# Autodesk Inventor assembly: L3 Gearbox Assembly
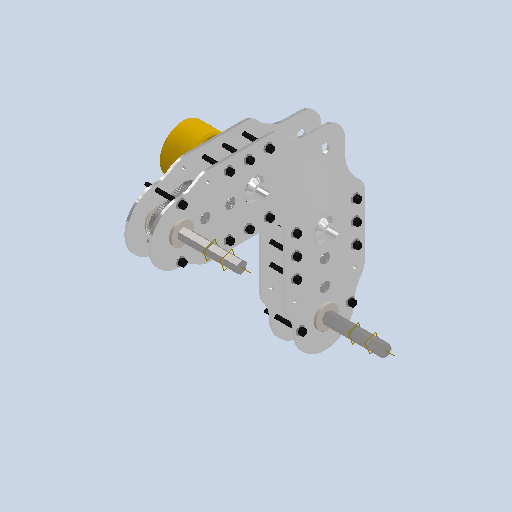
[picture p0: Inventor's stored thumbnail of the model, 512x512]
Saved by Autodesk Inventor 2025.1 (Build 291241020, 241B)
## iProperties
Created: 2023-02-14
Part Number: L3 Gearbox Assembly
Document SubType Name: Assembly
Designer: Dave
Mass: 1965.41 g
Surface Area: 3646.76 cm^2
Volume: 537.619 cm^3
Density: 3.65577 g/cm^3
Author: Dave
## Documents named in this file (15)
- C:\Users\t205b\OneDrive\Documents\Github\BehrendURCMechanical\CAD\Chassis V3\L3 Gearbox Assembly.iam
- C:\Users\t205b\OneDrive\Documents\Github\BehrendURCMechanical\CAD\Chassis\GearBox\Final Gears and Assemblies\CH-1-01-20T_Drive Gear.ipt
- C:\Users\t205b\OneDrive\Documents\Github\BehrendURCMechanical\CAD\Chassis\GearBox\Final Gears and Assemblies\CH-1-01-60T_Output.ipt
- C:\Users\t205b\OneDrive\Documents\Github\BehrendURCMechanical\CAD\Chassis\GearBox\Final Gears and Assemblies\CH-1-01-20T_Idler.ipt
- C:\Users\t205b\OneDrive\Documents\Github\BehrendURCMechanical\CAD\Chassis\GearBox\Final Gears and Assemblies\CH-1-01-60T_Idler.ipt
- C:\Users\t205b\OneDrive\Documents\Github\BehrendURCMechanical\CAD\Chassis\GearBox\Drive Motor Shaft Coupler.ipt
- C:\Users\t205b\OneDrive\Documents\Github\BehrendURCMechanical\CAD\Chassis\GearBox\Ch-1-01-0.5x4.5HexShaft.ipt
- C:\Users\t205b\OneDrive\Documents\Github\BehrendURCMechanical\CAD\Chassis\GearBox\CH-1-01-0.25x1.875SmoothShaft.ipt
- C:\Users\t205b\OneDrive\Documents\Github\BehrendURCMechanical\CAD\Chassis\GearBox\CH-1-01-0.5HexBearing.ipt
- C:\Users\t205b\OneDrive\Documents\Github\BehrendURCMechanical\CAD\Chassis\GearBox\CH-1-01-0.25IDSmoothBoreBearing.ipt
- C:\Users\t205b\OneDrive\Documents\Github\BehrendURCMechanical\CAD\Chassis V3\DriveMotorAssem\DriveMotorAssem.iam
- C:\Users\t205b\OneDrive\Documents\Github\BehrendURCMechanical\CAD\Chassis V3\91251A252_Black-Oxide Alloy Steel Socket Head Screw.ipt
- C:\Users\Dave\Downloads\91831A011_18-8 Stainless Steel Nylon-Insert Locknut (1).ipt
- C:\Users\t205b\OneDrive\Documents\Github\BehrendURCMechanical\CAD\Chassis V3\90107A011_316 Stainless Steel Washer.ipt
- C:\Users\t205b\OneDrive\Documents\Github\BehrendURCMechanical\CAD\Chassis V3\L3Plate.ipt
## Components (99 placed, 14 different names)
1. L3Plate:1 — Insert:13, Insert:14, Insert:15, Insert:16, Insert:17, Insert:18, Insert:19, Insert:20
2. L3Plate:2 — Mate:29, Insert:39, Insert:41
3. CH-1-01-0.25IDSmoothBoreBearing:4 — Mate:10, Mate:21
4. DriveMotorAssem:1 [sub-assembly] — Mate:27, Insert:21, Insert:22, Insert:23, Insert:24, Insert:25, Insert:26, Mate:29, Mate:30, Mate:31
5. 91831A011_18-8 Stainless Steel Nylon-Insert Locknut (1):4 — Insert:36
6. 91251A252_Black-Oxide Alloy Steel Socket Head Screw:1 — Insert:27, Mate:31
7. 90107A011_316 Stainless Steel Washer:1 — Insert:23, Insert:36
8. 91831A011_18-8 Stainless Steel Nylon-Insert Locknut (1):3 — Insert:37
9. 90107A011_316 Stainless Steel Washer:4 — Insert:22, Insert:37
10. 91251A252_Black-Oxide Alloy Steel Socket Head Screw:2 — Insert:28
11. 90107A011_316 Stainless Steel Washer:6 — Insert:21, Insert:38
12. 91251A252_Black-Oxide Alloy Steel Socket Head Screw:5 — Insert:30
13. 91831A011_18-8 Stainless Steel Nylon-Insert Locknut (1):2 — Insert:38
14. 91251A252_Black-Oxide Alloy Steel Socket Head Screw:6 — Insert:33
15. 91831A011_18-8 Stainless Steel Nylon-Insert Locknut (1):5 — Insert:42
16. 90107A011_316 Stainless Steel Washer:12 — Insert:24, Insert:42
17. 91251A252_Black-Oxide Alloy Steel Socket Head Screw:7 — Insert:34
18. 91831A011_18-8 Stainless Steel Nylon-Insert Locknut (1):6 — Insert:43
19. 90107A011_316 Stainless Steel Washer:14 — Insert:25, Insert:43
20. 91251A252_Black-Oxide Alloy Steel Socket Head Screw:8 — Insert:35
21. 91831A011_18-8 Stainless Steel Nylon-Insert Locknut (1):8 — Insert:44
22. 90107A011_316 Stainless Steel Washer:16 — Insert:26, Insert:44
23. 91251A252_Black-Oxide Alloy Steel Socket Head Screw:4 — Insert:32
24. 91831A011_18-8 Stainless Steel Nylon-Insert Locknut (1):7 — Insert:40
25. 90107A011_316 Stainless Steel Washer:10 — Insert:40, Insert:41
26. 91251A252_Black-Oxide Alloy Steel Socket Head Screw:3 — Insert:31
27. 91831A011_18-8 Stainless Steel Nylon-Insert Locknut (1):1 — Insert:45
28. 90107A011_316 Stainless Steel Washer:8 — Insert:39, Insert:45
29. CH-1-01-0.5HexBearing:1 — Mate:17, Flush:8
30. Ch-1-01-0.5x4.5HexShaft:1 — Mate:8, Mate:9, Flush:8
31. CH-1-01-0.25IDSmoothBoreBearing:3 — Flush:4, Mate:18, Mate:20, Mate:22, Mate:28
32. CH-1-01-0.25x1.875SmoothShaft:2 — Insert:12, Flush:4, Mate:28
33. Drive Motor Shaft Coupler:1 — Mate:27, Mate:30, Insert:29
34. CH-1-01-0.25IDSmoothBoreBearing:2 — Mate:11
35. CH-1-01-0.25x1.875SmoothShaft:1
36. CH-1-01-0.25IDSmoothBoreBearing:1 — Insert:12
37. CH-1-01-0.5HexBearing:2 — Mate:8, Mate:9
38. CH-1-01-20T_Drive Gear:1 — Insert:29
39. CH-1-01-60T_Idler:2 — Mate:10, Mate:11
40. CH-1-01-20T_Idler:1 — Mate:21, Flush:5
41. CH-1-01-60T_Idler:1 — Mate:18, Mate:19, Mate:20, Flush:5
42. CH-1-01-20T_Idler:2 — Mate:19, Mate:22, Flush:6
43. CH-1-01-60T_Output:1 — Mate:17, Flush:6
44. 90107A011_316 Stainless Steel Washer:11 — Insert:18, Insert:33
45. 90107A011_316 Stainless Steel Washer:13 — Insert:19, Insert:34
46. 90107A011_316 Stainless Steel Washer:15 — Insert:20, Insert:35
47. 90107A011_316 Stainless Steel Washer:9 — Insert:17, Insert:32
48. 90107A011_316 Stainless Steel Washer:7 — Insert:16, Insert:31
49. 90107A011_316 Stainless Steel Washer:5 — Insert:15, Insert:30
50. 90107A011_316 Stainless Steel Washer:3 — Insert:14, Insert:28
51. 90107A011_316 Stainless Steel Washer:2 — Insert:13, Insert:27
52. DriveMotorAssem:2 [sub-assembly]
53. 91831A011_18-8 Stainless Steel Nylon-Insert Locknut (1):9
54. 91251A252_Black-Oxide Alloy Steel Socket Head Screw:9
55. 90107A011_316 Stainless Steel Washer:17
56. 91831A011_18-8 Stainless Steel Nylon-Insert Locknut (1):10
57. 90107A011_316 Stainless Steel Washer:18
58. 91251A252_Black-Oxide Alloy Steel Socket Head Screw:10
59. 90107A011_316 Stainless Steel Washer:19
60. 91251A252_Black-Oxide Alloy Steel Socket Head Screw:11
61. 91831A011_18-8 Stainless Steel Nylon-Insert Locknut (1):11
62. 91251A252_Black-Oxide Alloy Steel Socket Head Screw:12
63. 91831A011_18-8 Stainless Steel Nylon-Insert Locknut (1):12
64. 90107A011_316 Stainless Steel Washer:20
65. 91251A252_Black-Oxide Alloy Steel Socket Head Screw:13
66. 91831A011_18-8 Stainless Steel Nylon-Insert Locknut (1):13
67. 90107A011_316 Stainless Steel Washer:21
68. 91251A252_Black-Oxide Alloy Steel Socket Head Screw:14
69. 91831A011_18-8 Stainless Steel Nylon-Insert Locknut (1):14
70. 90107A011_316 Stainless Steel Washer:22
71. 91251A252_Black-Oxide Alloy Steel Socket Head Screw:15
72. 91831A011_18-8 Stainless Steel Nylon-Insert Locknut (1):15
73. 90107A011_316 Stainless Steel Washer:23
74. 91251A252_Black-Oxide Alloy Steel Socket Head Screw:16
75. 91831A011_18-8 Stainless Steel Nylon-Insert Locknut (1):16
76. 90107A011_316 Stainless Steel Washer:24
77. CH-1-01-0.5HexBearing:3
78. Ch-1-01-0.5x4.5HexShaft:2
79. CH-1-01-0.25IDSmoothBoreBearing:5
80. CH-1-01-0.25x1.875SmoothShaft:3
81. Drive Motor Shaft Coupler:2
82. CH-1-01-0.25IDSmoothBoreBearing:6
83. CH-1-01-0.25x1.875SmoothShaft:4
84. CH-1-01-0.25IDSmoothBoreBearing:7
85. CH-1-01-0.5HexBearing:4
86. CH-1-01-20T_Drive Gear:2
87. CH-1-01-60T_Idler:3
88. CH-1-01-20T_Idler:3
89. CH-1-01-60T_Idler:4
90. CH-1-01-20T_Idler:4
91. CH-1-01-60T_Output:2
92. 90107A011_316 Stainless Steel Washer:25
93. 90107A011_316 Stainless Steel Washer:26
94. 90107A011_316 Stainless Steel Washer:27
95. 90107A011_316 Stainless Steel Washer:28
96. 90107A011_316 Stainless Steel Washer:29
97. 90107A011_316 Stainless Steel Washer:30
98. 90107A011_316 Stainless Steel Washer:31
99. 90107A011_316 Stainless Steel Washer:32
## Component patterns: (2 elements, first: DriveMotorAssem:1 + 91831A011_18-8 Stainless Steel Nylon-Insert Locknut (1):4 + 91251A252_Black-Oxide Alloy Steel Socket Head Screw:1 + 90107A011_316 Stainless Steel Washer:1 + 91831A011_18-8 Stainless Steel Nylon-Insert Locknut (1):3 + 90107A011_316 Stainless Steel Washer:4 + 91251A252_Black-Oxide Alloy Steel Socket Head Screw:2 + 90107A011_316 Stainless Steel Washer:6 + 91251A252_Black-Oxide Alloy Steel Socket Head Screw:5 + 91831A011_18-8 Stainless Steel Nylon-Insert Locknut (1):2 + 91251A252_Black-Oxide Alloy Steel Socket Head Screw:6 + 91831A011_18-8 Stainless Steel Nylon-Insert Locknut (1):5 + 90107A011_316 Stainless Steel Washer:12 + 91251A252_Black-Oxide Alloy Steel Socket Head Screw:7 + 91831A011_18-8 Stainless Steel Nylon-Insert Locknut (1):6 + 90107A011_316 Stainless Steel Washer:14 + 91251A252_Black-Oxide Alloy Steel Socket Head Screw:8 + 91831A011_18-8 Stainless Steel Nylon-Insert Locknut (1):8 + 90107A011_316 Stainless Steel Washer:16 + 91251A252_Black-Oxide Alloy Steel Socket Head Screw:4 + 91831A011_18-8 Stainless Steel Nylon-Insert Locknut (1):7 + 90107A011_316 Stainless Steel Washer:10 + 91251A252_Black-Oxide Alloy Steel Socket Head Screw:3 + 91831A011_18-8 Stainless Steel Nylon-Insert Locknut (1):1 + 90107A011_316 Stainless Steel Washer:8 + CH-1-01-0.5HexBearing:1 + Ch-1-01-0.5x4.5HexShaft:1 + CH-1-01-0.25IDSmoothBoreBearing:3 + CH-1-01-0.25x1.875SmoothShaft:2 + Drive Motor Shaft Coupler:1 + CH-1-01-0.25IDSmoothBoreBearing:2 + CH-1-01-0.25x1.875SmoothShaft:1 + CH-1-01-0.25IDSmoothBoreBearing:1 + CH-1-01-0.5HexBearing:2 + CH-1-01-20T_Drive Gear:1 + CH-1-01-60T_Idler:2 + CH-1-01-20T_Idler:1 + CH-1-01-60T_Idler:1 + CH-1-01-20T_Idler:2 + CH-1-01-60T_Output:1 + 90107A011_316 Stainless Steel Washer:11 + 90107A011_316 Stainless Steel Washer:13 + 90107A011_316 Stainless Steel Washer:15 + 90107A011_316 Stainless Steel Washer:9 + 90107A011_316 Stainless Steel Washer:7 + 90107A011_316 Stainless Steel Washer:5 + 90107A011_316 Stainless Steel Washer:3 + 90107A011_316 Stainless Steel Washer:2)
## Relationships (62: Insert 40, Mate 16, Flush 5, Angle 1)
- [Angle] (0 deg): L3Plate:1
- [Flush]: L3Plate:1 ↔ L3Plate:2
- [Insert]: L3Plate:1 ↔ CH-1-01-0.25IDSmoothBoreBearing:1
- [Insert]: L3Plate:1 ↔ CH-1-01-0.25IDSmoothBoreBearing:2
- [Insert]: L3Plate:2 ↔ CH-1-01-0.25IDSmoothBoreBearing:3
- [Insert]: L3Plate:2 ↔ CH-1-01-0.25IDSmoothBoreBearing:4
- [Insert]: L3Plate:1 ↔ CH-1-01-0.5HexBearing:2
- [Insert]: L3Plate:2 ↔ CH-1-01-0.5HexBearing:1
- Mate:8: Ch-1-01-0.5x4.5HexShaft:1 ↔ CH-1-01-0.5HexBearing:2
- Mate:9: Ch-1-01-0.5x4.5HexShaft:1 ↔ CH-1-01-0.5HexBearing:2
- Insert:12: CH-1-01-0.25x1.875SmoothShaft:2 ↔ CH-1-01-0.25IDSmoothBoreBearing:1
- Mate:10: CH-1-01-0.25IDSmoothBoreBearing:4 ↔ CH-1-01-60T_Idler:2
- Mate:11: CH-1-01-0.25IDSmoothBoreBearing:2 ↔ CH-1-01-60T_Idler:2
- Flush:4: CH-1-01-0.25IDSmoothBoreBearing:3 ↔ CH-1-01-0.25x1.875SmoothShaft:2
- Mate:17: CH-1-01-0.5HexBearing:1 ↔ CH-1-01-60T_Output:1
- Mate:18: CH-1-01-0.25IDSmoothBoreBearing:3 ↔ CH-1-01-60T_Idler:1
- Mate:19: CH-1-01-60T_Idler:1 ↔ CH-1-01-20T_Idler:2
- Mate:20: CH-1-01-0.25IDSmoothBoreBearing:3 ↔ CH-1-01-60T_Idler:1
- Mate:21: CH-1-01-0.25IDSmoothBoreBearing:4 ↔ CH-1-01-20T_Idler:1
- Flush:5: CH-1-01-20T_Idler:1 ↔ CH-1-01-60T_Idler:1
- Mate:22: CH-1-01-0.25IDSmoothBoreBearing:3 ↔ CH-1-01-20T_Idler:2
- Flush:6: CH-1-01-20T_Idler:2 ↔ CH-1-01-60T_Output:1
- Flush:8: CH-1-01-0.5HexBearing:1 ↔ Ch-1-01-0.5x4.5HexShaft:1
- [Mate]: L3Plate:1 ↔ Drive Motor Shaft Coupler:1
- Mate:27: DriveMotorAssem:1 ↔ Drive Motor Shaft Coupler:1
- Mate:28: CH-1-01-0.25IDSmoothBoreBearing:3 ↔ CH-1-01-0.25x1.875SmoothShaft:2
- Insert:13: L3Plate:1 ↔ 90107A011_316 Stainless Steel Washer:2
- Insert:14: L3Plate:1 ↔ 90107A011_316 Stainless Steel Washer:3
- Insert:15: L3Plate:1 ↔ 90107A011_316 Stainless Steel Washer:5
- Insert:16: L3Plate:1 ↔ 90107A011_316 Stainless Steel Washer:7
- Insert:17: L3Plate:1 ↔ 90107A011_316 Stainless Steel Washer:9
- Insert:18: L3Plate:1 ↔ 90107A011_316 Stainless Steel Washer:11
- Insert:19: L3Plate:1 ↔ 90107A011_316 Stainless Steel Washer:13
- Insert:20: L3Plate:1 ↔ 90107A011_316 Stainless Steel Washer:15
- Insert:21: DriveMotorAssem:1 ↔ 90107A011_316 Stainless Steel Washer:6
- Insert:22: DriveMotorAssem:1 ↔ 90107A011_316 Stainless Steel Washer:4
- Insert:23: DriveMotorAssem:1 ↔ 90107A011_316 Stainless Steel Washer:1
- Insert:24: DriveMotorAssem:1 ↔ 90107A011_316 Stainless Steel Washer:12
- Insert:25: DriveMotorAssem:1 ↔ 90107A011_316 Stainless Steel Washer:14
- Insert:26: DriveMotorAssem:1 ↔ 90107A011_316 Stainless Steel Washer:16
- Insert:27: 91251A252_Black-Oxide Alloy Steel Socket Head Screw:1 ↔ 90107A011_316 Stainless Steel Washer:2
- Insert:28: 91251A252_Black-Oxide Alloy Steel Socket Head Screw:2 ↔ 90107A011_316 Stainless Steel Washer:3
- Mate:29: L3Plate:2 ↔ DriveMotorAssem:1
- Mate:30: DriveMotorAssem:1 ↔ Drive Motor Shaft Coupler:1
- Insert:29: Drive Motor Shaft Coupler:1 ↔ CH-1-01-20T_Drive Gear:1
- Insert:30: 91251A252_Black-Oxide Alloy Steel Socket Head Screw:5 ↔ 90107A011_316 Stainless Steel Washer:5
- Insert:31: 91251A252_Black-Oxide Alloy Steel Socket Head Screw:3 ↔ 90107A011_316 Stainless Steel Washer:7
- Insert:32: 91251A252_Black-Oxide Alloy Steel Socket Head Screw:4 ↔ 90107A011_316 Stainless Steel Washer:9
- Insert:33: 91251A252_Black-Oxide Alloy Steel Socket Head Screw:6 ↔ 90107A011_316 Stainless Steel Washer:11
- Insert:34: 91251A252_Black-Oxide Alloy Steel Socket Head Screw:7 ↔ 90107A011_316 Stainless Steel Washer:13
- Insert:35: 91251A252_Black-Oxide Alloy Steel Socket Head Screw:8 ↔ 90107A011_316 Stainless Steel Washer:15
- Mate:31: DriveMotorAssem:1 ↔ 91251A252_Black-Oxide Alloy Steel Socket Head Screw:1
- Insert:36: 91831A011_18-8 Stainless Steel Nylon-Insert Locknut (1):4 ↔ 90107A011_316 Stainless Steel Washer:1
- Insert:37: 91831A011_18-8 Stainless Steel Nylon-Insert Locknut (1):3 ↔ 90107A011_316 Stainless Steel Washer:4
- Insert:38: 90107A011_316 Stainless Steel Washer:6 ↔ 91831A011_18-8 Stainless Steel Nylon-Insert Locknut (1):2
- Insert:39: L3Plate:2 ↔ 90107A011_316 Stainless Steel Washer:8
- Insert:40: 91831A011_18-8 Stainless Steel Nylon-Insert Locknut (1):7 ↔ 90107A011_316 Stainless Steel Washer:10
- Insert:41: L3Plate:2 ↔ 90107A011_316 Stainless Steel Washer:10
- Insert:42: 91831A011_18-8 Stainless Steel Nylon-Insert Locknut (1):5 ↔ 90107A011_316 Stainless Steel Washer:12
- Insert:43: 91831A011_18-8 Stainless Steel Nylon-Insert Locknut (1):6 ↔ 90107A011_316 Stainless Steel Washer:14
- Insert:44: 91831A011_18-8 Stainless Steel Nylon-Insert Locknut (1):8 ↔ 90107A011_316 Stainless Steel Washer:16
- Insert:45: 91831A011_18-8 Stainless Steel Nylon-Insert Locknut (1):1 ↔ 90107A011_316 Stainless Steel Washer:8
